# Autodesk Inventor assembly: Assy_fork_right
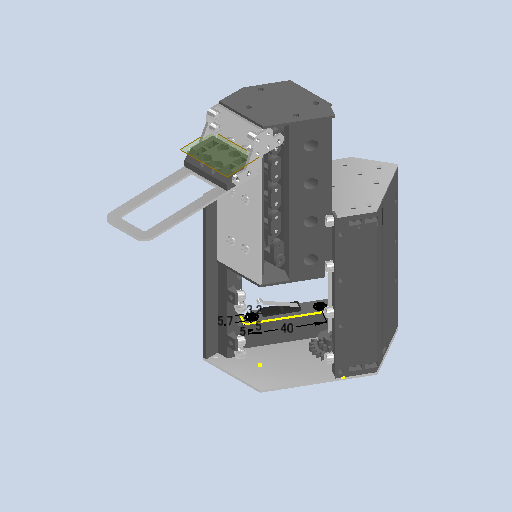
[picture p0: Inventor's stored thumbnail of the model, 512x512]
Saved by Autodesk Inventor 2024.1 (Build 281209000, 209)
## iProperties
Created: 2025-01-17
Part Number: Assy_fork_right
Document SubType Name: Assembly
Designer: hibik
Author: hibik
## Documents named in this file (6)
- C:\Users\hibik\Documents\Robomech\RESCUE\ORCA\hard\fork\right\Assy_fork_right.iam
- C:\Users\hibik\Documents\Robomech\RESCUE\ORCA\hard\fork\right\base_wall_added.iam
- C:\Users\hibik\Documents\Robomech\RESCUE\ORCA\hard\fork\right\screw.iam
- C:\Users\hibik\Documents\Robomech\RESCUE\ORCA\hard\fork\right\rail.iam
- C:\Users\hibik\Documents\Robomech\RESCUE\ORCA\hard\fork\right\motor_set.iam
- C:\Users\hibik\Documents\Robomech\RESCUE\ORCA\hard\fork\right\screw_gear_under_12.ipt
## Components (5 placed, 5 different names)
1. base_wall_added:1 [sub-assembly] — 挿入:1, 正接:1, 正接:2, 正接:3, 正接:4, 挿入:2, 角度:1, 挿入:3
2. screw:1 [sub-assembly] — 挿入:1
3. rail:1 [sub-assembly] — 正接:1, 正接:2, 正接:3, 正接:4
4. motor_set:1 [sub-assembly] — 挿入:2, 角度:1
5. screw_gear_under_12:1 — 挿入:3
## Relationships (8: Tangent 4, Insert 3, Angle 1)
- 挿入:1 [Insert]: base_wall_added:1 ↔ screw:1
- 正接:1 [Tangent]: base_wall_added:1 ↔ rail:1
- 正接:2 [Tangent]: base_wall_added:1 ↔ rail:1
- 正接:3 [Tangent]: base_wall_added:1 ↔ rail:1
- 正接:4 [Tangent]: base_wall_added:1 ↔ rail:1
- 挿入:2 [Insert]: base_wall_added:1 ↔ motor_set:1
- 角度:1 [Angle] (0 deg): base_wall_added:1 ↔ motor_set:1
- 挿入:3 [Insert]: base_wall_added:1 ↔ screw_gear_under_12:1
